# Autodesk Inventor assembly: Estructura 1617045494032
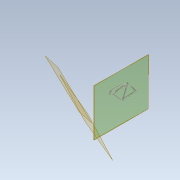
[picture p0: Inventor's stored thumbnail of the model, 180x180]
Saved by Autodesk Inventor 2021 (Build 250183000, 183)
## iProperties
_FrameDoc: Frame Assembly
_Version: 25.0.0
Created: 2021-03-29
Part Number: Estructura 1617045494032
Document SubType Name: Assembly
Designer: j2seb
Author: j2seb
## Documents named in this file (17)
- C:\Git\Proyecto_APM\02 Inventor\Marco_Bicicleta\Frame\Estructura 1617045494032.iam
- C:\Git\Proyecto_APM\02 Inventor\Marco_Bicicleta\Frame\Skeleton 1617045494196.ipt
- C:\Git\Proyecto_APM\02 Inventor\Marco_Bicicleta\Frame\ANSI  1617061821453.ipt
- C:\Git\Proyecto_APM\02 Inventor\Marco_Bicicleta\Frame\ANSI  1617061275537.ipt
- ANSI  1617061275537.ipt
- C:\Git\Proyecto_APM\02 Inventor\Marco_Bicicleta\Frame\ANSI  1617061428950.ipt
- ANSI  1617061428950.ipt
- C:\Git\Proyecto_APM\02 Inventor\Marco_Bicicleta\Frame\ANSI  1617061469895.ipt
- C:\Git\Proyecto_APM\02 Inventor\Marco_Bicicleta\Frame\ANSI  1617061519425.ipt
- ANSI  1617061519425.ipt
- C:\Git\Proyecto_APM\02 Inventor\Marco_Bicicleta\Frame\ANSI  1617061763005.ipt
- ANSI  1617061763005.ipt
- C:\Git\Proyecto_APM\02 Inventor\Marco_Bicicleta\Frame\ANSI  1617061857590.ipt
- ANSI  1617061857590.ipt
- C:\Git\Proyecto_APM\02 Inventor\Marco_Bicicleta\Frame\ANSI  1617061874634.ipt
- ANSI  1617061874634.ipt
- C:\Git\Proyecto_APM\02 Inventor\Marco_Bicicleta\Frame\ANSI  1618003984630.ipt
## Components (10 placed, 10 different names)
1. Skeleton 1617045494196:1
2. ANSI  1617061428950:1
3. ANSI  1617061275537:1
4. ANSI  1617061763005:1 — Nivelación:1
5. ANSI  1617061857590:1
6. ANSI  1617061874634:1
7. ANSI  1617061519425:1
8. ANSI  1617061821453:1
9. ANSI  1617061469895:1
10. ANSI  1618003984630:1 — Nivelación:1
## Relationships (1: Flush 1)
- Nivelación:1 [Flush]: ANSI  1617061763005:1 ↔ ANSI  1618003984630:1
